# Autodesk Inventor assembly: stackedSpool
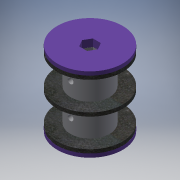
[picture p0: Inventor's stored thumbnail of the model, 180x180]
Saved by Autodesk Inventor 2019.3 (Build 233278000, 278)
## iProperties
Created: 2019-03-05
Part Number: stackedSpool
Document SubType Name: Assembly
Designer: steele
Author: steele
## Documents named in this file (4)
- C:\git\CAD-Development\robSteele\RevRoboticsExtrusionAttachements\stackedSpool.iam
- C:\git\CAD-Development\robSteele\RevRoboticsExtrusionAttachements\spacerForEnd.ipt
- C:\git\CAD-Development\robSteele\RevRoboticsExtrusionAttachements\washer2_5x1_0.ipt
- C:\git\CAD-Development\robSteele\RevRoboticsExtrusionAttachements\spoolV03.ipt
## Components (7 placed, 3 different names)
1. spacerForEnd:1 — Insert:1
2. washer2_5x1_0:1 — Insert:1, Insert:2
3. spoolV03:1 — Insert:2, Insert:3
4. washer2_5x1_0:2 — Insert:3, Insert:4
5. spoolV03:2 — Insert:4, Insert:5
6. washer2_5x1_0:3 — Insert:5, Insert:6
7. spacerForEnd:2 — Insert:6
## Relationships (6: Insert 6)
- Insert:1: spacerForEnd:1 ↔ washer2_5x1_0:1
- Insert:2: washer2_5x1_0:1 ↔ spoolV03:1
- Insert:3: spoolV03:1 ↔ washer2_5x1_0:2
- Insert:4: washer2_5x1_0:2 ↔ spoolV03:2
- Insert:5: spoolV03:2 ↔ washer2_5x1_0:3
- Insert:6: washer2_5x1_0:3 ↔ spacerForEnd:2
